# Autodesk Inventor assembly: Rack and Pinion-Drive
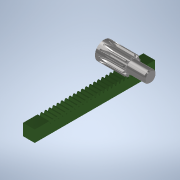
[picture p0: Inventor's stored thumbnail of the model, 180x180]
Saved by Autodesk Inventor 2022 (Build 260153000, 153)
## iProperties
Created: 2013-11-13
Part Number: Rack and Pinion-Drive
Document SubType Name: Assembly
Designer: NiveshandNisheeth
Author: NiveshandNisheeth
## Documents named in this file (3)
- F:\Temp\Call of Duty - Black Ops\rack-and-pinion-pinhao-cremalheira-1.snapshot.2\Rack and Pinion-Drive.iam
- F:\Temp\Call of Duty - Black Ops\rack-and-pinion-pinhao-cremalheira-1.snapshot.2\PINION.ipt
- F:\Temp\Call of Duty - Black Ops\rack-and-pinion-pinhao-cremalheira-1.snapshot.2\RACK.ipt
## Components (2 placed, 2 different names)
1. PINION:1 — Mate:1, Mate:2, Tangent:1, Mate:3, Drive, Rotation/Translation:1
2. RACK:1 — Tangent:1, Angle:1, Mate:3, Rotation/Translation:1
## Relationships (7: Mate 3, Angle 2, Tangent 1, RelateRotateTranslate 1)
- Mate:1: PINION:1
- Mate:2: PINION:1
- Tangent:1: PINION:1 ↔ RACK:1
- Angle:1 (0 deg): RACK:1
- Mate:3: PINION:1 ↔ RACK:1
- Drive [Angle] (0 deg): PINION:1
- Rotation/Translation:1 [RelateRotateTranslate] (120.015 mm): PINION:1 ↔ RACK:1
